# Autodesk Inventor assembly: Assembly2
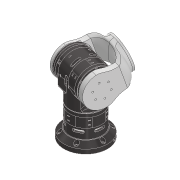
[picture p0: Inventor's stored thumbnail of the model, 180x180]
Saved by Autodesk Inventor 2021 (Build 250183000, 183)
## iProperties
Created: 2020-08-06
Part Number: Assembly2
Document SubType Name: Assembly
Designer: Derm
Author: Derm
## Documents named in this file (5)
- C:\Users\Derm\roboticArm\hardware\v9\Assembly2.iam
- C:\Users\Derm\roboticArm\hardware\v9\j0.iam
- C:\Users\Derm\roboticArm\hardware\v9\j1.iam
- C:\Users\Derm\roboticArm\hardware\v9\j1Housing.ipt
- C:\Users\Derm\roboticArm\hardware\v9\upperArmMain.ipt
## Components (4 placed, 4 different names)
1. j0:1 [sub-assembly] — Mate:1, Mate:2, Mate:3, Mate:4, Angle:1, Mate:5, Mate:6
2. j1:1 [sub-assembly] — Mate:2, Mate:3, Mate:6, Mate:7, Mate:8
3. j1Housing:1 — Mate:4, Angle:1, Mate:5
4. upperArmMain:1 — Mate:7, Mate:8
## Relationships (9: Mate 8, Angle 1)
- Mate:1: j0:1
- Mate:2: j0:1 ↔ j1:1
- Mate:3: j0:1 ↔ j1:1
- Mate:4: j0:1 ↔ j1Housing:1
- Angle:1 (0 deg): j0:1 ↔ j1Housing:1
- Mate:5: j0:1 ↔ j1Housing:1
- Mate:6: j0:1 ↔ j1:1
- Mate:7: j1:1 ↔ upperArmMain:1
- Mate:8: j1:1 ↔ upperArmMain:1
